# Autodesk Inventor assembly: hashikadai1
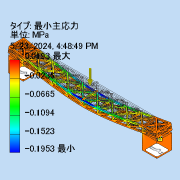
[picture p0: Inventor's stored thumbnail of the model, 180x180]
Saved by Autodesk Inventor 2022 (Build 260153000, 153)
## iProperties
Created: 2024-05-14
Part Number: hashikadai1
Document SubType Name: Assembly
Designer: ktamu
Author: ktamu
## Documents named in this file (10)
- D:\SDinventor\DesignHashi\DesignHashi3kintouNNNNzure\hashikadai1.iam
- D:\SDinventor\DesignHashi\DesignHashi3kintouNNNNzure\hashgeta1.ipt
- D:\SDinventor\DesignHashi\DesignHashi3kintouNNNNzure\hashi1shado.ipt
- D:\SDinventor\DesignHashi\DesignHashi3kintouNNNNzure\loadstick.ipt
- D:\SDinventor\DesignHashi\DesignHashi3kintouNNNNzure\hashikadai1\AIP\FEA\ep6vs5l7k.ftes
- D:\SDinventor\DesignHashi\DesignHashi3kintouNNNNzure\hashikadai1\AIP\FEA\ep6vs5l7k.fwiz
- D:\SDinventor\DesignHashi\DesignHashi3kintouNNNNzure\hashikadai1\AIP\FEA\ep6vs5l9c.fmsh
- D:\SDinventor\DesignHashi\DesignHashi3kintouNNNNzure\hashikadai1\AIP\FEA\ep6vs5l9d.fres
- D:\SDinventor\DesignHashi\DesignHashi3kintouNNNNzure\hashikadai1\AIP\FEA\ep6vs5l7k.fins
- D:\SDinventor\DesignHashi\DesignHashi3kintouNNNNzure\hashikadai1\AIP\FEA\ep6vs5l7k.fsat
## Components (4 placed, 3 different names)
1. hashgeta1:1 — メイト:1, フラッシュ:1, フラッシュ:2
2. hashi1shado:1 — メイト:1, フラッシュ:1, フラッシュ:2, フラッシュ:3, フラッシュ:4, メイト:2, フラッシュ:5, メイト:3
3. hashgeta1:2 — フラッシュ:3, フラッシュ:4, メイト:2, フラッシュ:6
4. loadstick:1 — フラッシュ:5, メイト:3, フラッシュ:6
## Relationships (9: Flush 6, Mate 3)
- メイト:1 [Mate]: hashgeta1:1 ↔ hashi1shado:1
- フラッシュ:1 [Flush]: hashgeta1:1 ↔ hashi1shado:1
- フラッシュ:2 [Flush]: hashgeta1:1 ↔ hashi1shado:1
- フラッシュ:3 [Flush]: hashi1shado:1 ↔ hashgeta1:2
- フラッシュ:4 [Flush]: hashi1shado:1 ↔ hashgeta1:2
- メイト:2 [Mate]: hashi1shado:1 ↔ hashgeta1:2
- フラッシュ:5 [Flush]: hashi1shado:1 ↔ loadstick:1
- メイト:3 [Mate]: hashi1shado:1 ↔ loadstick:1
- フラッシュ:6 [Flush] (248 mm): hashgeta1:2 ↔ loadstick:1
